# Autodesk Inventor assembly: Assembly3
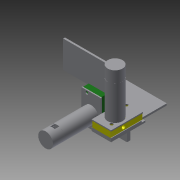
[picture p0: Inventor's stored thumbnail of the model, 180x180]
Saved by Autodesk Inventor 2015 SP1 (Build 190203100, 203)
## iProperties
Created: 2015-06-10
Part Number: Assembly3
Document SubType Name: Assembly
Designer: pc
Author: pc
## Documents named in this file (7)
- C:\Users\pc\Desktop\sensores.diametro\juntas\Assembly3.iam
- C:\Users\pc\Desktop\sensores.diametro\juntas\soporte.ipt
- C:\Users\pc\Desktop\sensores.diametro\juntas\tapaA0.2.ipt
- C:\Users\pc\Desktop\sensores.diametro\juntas\tapaB0.2.ipt
- C:\Users\pc\Desktop\sensores.diametro\juntas\TORRE.ipt
- C:\Users\pc\Desktop\sensores.diametro\juntas\capuchon.torre.ipt
- C:\Users\pc\Desktop\sensores.diametro\Horizontal\sensores.ipt
## Components (9 placed, 6 different names)
1. soporte:1 — Insert:1, Insert:2, Insert:3, Insert:4, Mate:1, Mate:2, Mate:3, Mate:4, Mate:5, Mate:6
2. tapaA0.2:1 — Insert:1, Insert:2, Insert:5
3. tapaB0.2:1 — Insert:3, Insert:4, Insert:6
4. TORRE:1 — Insert:5, Insert:8
5. TORRE:2 — Insert:6, Insert:7
6. capuchon.torre:1 — Insert:7
7. capuchon.torre:2 — Insert:8
8. sensores:1 — Mate:1, Mate:2, Mate:3
9. sensores:2 — Mate:4, Mate:5, Mate:6
## Relationships (14: Insert 8, Mate 6)
- Insert:1 (1.5 mm): soporte:1 ↔ tapaA0.2:1
- Insert:2 (1.5 mm): soporte:1 ↔ tapaA0.2:1
- Insert:3 (1.5 mm): soporte:1 ↔ tapaB0.2:1
- Insert:4 (1.5 mm): soporte:1 ↔ tapaB0.2:1
- Insert:5: tapaA0.2:1 ↔ TORRE:1
- Insert:6: tapaB0.2:1 ↔ TORRE:2
- Insert:7: TORRE:2 ↔ capuchon.torre:1
- Insert:8: TORRE:1 ↔ capuchon.torre:2
- Mate:1: soporte:1 ↔ sensores:1
- Mate:2 (0.5 mm): soporte:1 ↔ sensores:1
- Mate:3: soporte:1 ↔ sensores:1
- Mate:4: soporte:1 ↔ sensores:2
- Mate:5 (0.5 mm): soporte:1 ↔ sensores:2
- Mate:6: soporte:1 ↔ sensores:2
